# Autodesk Inventor assembly: Assembly1
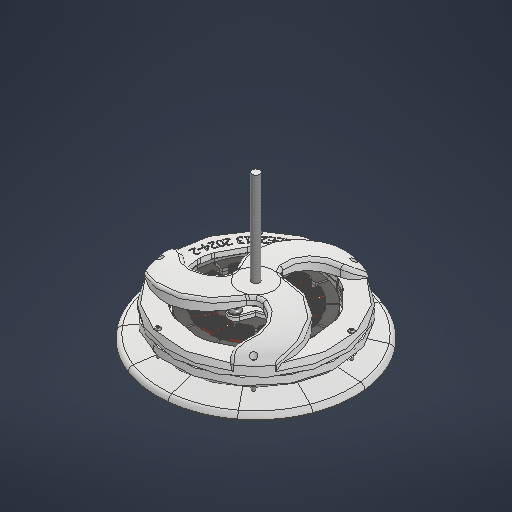
[picture p0: Inventor's stored thumbnail of the model, 512x512]
Saved by Autodesk Inventor 2025 (Build 290162010, 162A)
## iProperties
Created: 2024-11-09
Part Number: Assembly1
Document SubType Name: Assembly
Designer: river
Author: river
## Documents named in this file (15)
- C:\DATA\sem_08\Maquinas\proyecto\3d\Assembly1.iam
- C:\DATA\sem_08\Maquinas\proyecto\3d\lamina_estator.ipt
- C:\Users\river\Documents\Inventor\Content Center Files\R2025\en-US\DIN 625 SKF(4)\DIN 625 SKF - SKF 608-2Z.ipt
- C:\DATA\sem_08\Maquinas\proyecto\3d\perno.ipt
- C:\DATA\sem_08\Maquinas\proyecto\3d\lamina_rotor.ipt
- C:\DATA\sem_08\Maquinas\proyecto\3d\iman.ipt
- C:\DATA\sem_08\Maquinas\proyecto\3d\coil.ipt
- C:\DATA\sem_08\Maquinas\proyecto\3d\shell_b.ipt
- C:\DATA\sem_08\Maquinas\proyecto\3d\shell_t.ipt
- C:\Users\river\Documents\Inventor\Content Center Files\R2025\en-US\ANSI B18.3.4M(2)\ANSI B18.3.4M - M6 x 1 x 30(1).ipt
- C:\Users\river\Documents\Inventor\Content Center Files\R2025\en-US\ANSI B18.16.3M(2)\ANSI B18.16.3M - Property Class 5 and 10 - Metric M6 x 1 Metal Type.ipt
- C:\DATA\sem_08\Maquinas\proyecto\3d\rodamiento_t.ipt
- C:\DATA\sem_08\Maquinas\proyecto\3d\rodamiento_b.ipt
- C:\Users\river\Documents\Inventor\Content Center Files\R2025\en-US\ANSI B18.3.4M(2)\ANSI B18.3.4M - M3 x 0.5 x 25(1).ipt
- C:\Users\river\Documents\Inventor\Content Center Files\R2025\en-US\JIS B 1181 F C (1)\JIS B 1181 - M3(7).ipt
## Components (55 placed, 14 different names)
1. rodamiento_b:1 — Insert:19, Cylindrical:1, Insert:21
2. lamina_estator:1 — Mate:1, Mate:2, Flush:1, Insert:1, Flush:2
3. lamina_estator:2 — Insert:1, Flush:2, Insert:2, Flush:3, Mate:7
4. lamina_estator:3 — Insert:2, Flush:3, Insert:4, Insert:5, Insert:10, Mate:9
5. DIN 625 SKF- with two Z shields SKF 608-2Z:1 — Insert:3, Insert:9
6. DIN 625 SKF- with two Z shields SKF 608-2Z:2 — Insert:3, Insert:8
7. rodamiento_t:1 — Insert:4, Insert:5, Insert:8, Insert:14, Insert:19
8. perno:1 — Insert:9
9. lamina_rotor:1 — Mate:3, Flush:4, Flush:5, Insert:16, Mate:10
10. lamina_rotor:2 — Mate:3, Flush:4, Flush:5, Mate:4, Flush:6, Flush:7, Mate:5, Mate:6
11. lamina_rotor:3 — Mate:4, Flush:6, Flush:7, Insert:10
12. shell_t:1 — Insert:17, Insert:18, Insert:22
13. shell_b:1 — Insert:16, Mate:10, Insert:17, Insert:18, Insert:23
14. Prevailing Torque Type Hex Nut - Steel Metric Property Class 5 and 10 - Metric M6 x 1 Metal Type:1 — Insert:21
15. Forged Hexagon Socket Button Head Cap Screw - Metric M6 x 1 x 30:1 — Insert:14, Cylindrical:1
16. Prevailing Torque Type Hex Nut - Steel Metric Property Class 5 and 10 - Metric M6 x 1 Metal Type:2
17. Forged Hexagon Socket Button Head Cap Screw - Metric M6 x 1 x 30:2
18. Prevailing Torque Type Hex Nut - Steel Metric Property Class 5 and 10 - Metric M6 x 1 Metal Type:3
19. Forged Hexagon Socket Button Head Cap Screw - Metric M6 x 1 x 30:3
20. Prevailing Torque Type Hex Nut - Steel Metric Property Class 5 and 10 - Metric M6 x 1 Metal Type:4
21. Forged Hexagon Socket Button Head Cap Screw - Metric M6 x 1 x 30:4
22. Forged Hexagon Socket Button Head Cap Screw - Metric M3 x 0.5 x 25:1 — Insert:22
23. Forged Hexagon Socket Button Head Cap Screw - Metric M3 x 0.5 x 25:2
24. Forged Hexagon Socket Button Head Cap Screw - Metric M3 x 0.5 x 25:3
25. Forged Hexagon Socket Button Head Cap Screw - Metric M3 x 0.5 x 25:4
26. Forged Hexagon Socket Button Head Cap Screw - Metric M3 x 0.5 x 25:5
27. Forged Hexagon Socket Button Head Cap Screw - Metric M3 x 0.5 x 25:6
28. JIS B 1181 -finished Class 1 - Metric Class 1 -finishedM3:1 — Insert:23
29. JIS B 1181 -finished Class 1 - Metric Class 1 -finishedM3:2
30. JIS B 1181 -finished Class 1 - Metric Class 1 -finishedM3:3
31. JIS B 1181 -finished Class 1 - Metric Class 1 -finishedM3:4
32. JIS B 1181 -finished Class 1 - Metric Class 1 -finishedM3:5
33. JIS B 1181 -finished Class 1 - Metric Class 1 -finishedM3:6
34. coil:1 — Mate:7, Mate:9
35. coil:2
36. coil:3
37. coil:4
38. coil:5
39. coil:6
40. coil:7
41. coil:8
42. coil:9
43. coil:10
44. coil:11
45. coil:12
46. iman:1 — Mate:5, Mate:6
47. iman:2
48. iman:3
49. iman:4
50. iman:5
51. iman:6
52. iman:7
53. iman:8
54. iman:9
55. iman:10
## Component patterns: (4 elements, first: Prevailing Torque Type Hex Nut - Steel Metric Property Class 5 and 10 - Metric M6 x 1 Metal Type:1 + Forged Hexagon Socket Button Head Cap Screw - Metric M6 x 1 x 30:1), (6 elements, first: Forged Hexagon Socket Button Head Cap Screw - Metric M3 x 0.5 x 25:1), (6 elements, first: JIS B 1181 -finished Class 1 - Metric Class 1 -finishedM3:1), (12 elements, first: coil:1), (10 elements, first: iman:1)
## Relationships (33: Insert 16, Mate 9, Flush 7, CylindricalJoint 1)
- Mate:1: lamina_estator:1
- Mate:2: lamina_estator:1
- Flush:1: lamina_estator:1
- Insert:1: lamina_estator:1 ↔ lamina_estator:2
- Flush:2: lamina_estator:1 ↔ lamina_estator:2
- Insert:2: lamina_estator:2 ↔ lamina_estator:3
- Flush:3: lamina_estator:2 ↔ lamina_estator:3
- Insert:3: DIN 625 SKF- with two Z shields SKF 608-2Z:1 ↔ DIN 625 SKF- with two Z shields SKF 608-2Z:2
- Insert:4: lamina_estator:3 ↔ rodamiento_t:1
- Insert:5: lamina_estator:3 ↔ rodamiento_t:1
- Insert:8: DIN 625 SKF- with two Z shields SKF 608-2Z:2 ↔ rodamiento_t:1
- Insert:9: DIN 625 SKF- with two Z shields SKF 608-2Z:1 ↔ perno:1
- Mate:3: lamina_rotor:1 ↔ lamina_rotor:2
- Flush:4: lamina_rotor:1 ↔ lamina_rotor:2
- Flush:5: lamina_rotor:1 ↔ lamina_rotor:2
- Mate:4: lamina_rotor:2 ↔ lamina_rotor:3
- Flush:6: lamina_rotor:2 ↔ lamina_rotor:3
- Flush:7: lamina_rotor:2 ↔ lamina_rotor:3
- Insert:10: lamina_estator:3 ↔ lamina_rotor:3
- Mate:5: lamina_rotor:2 ↔ iman:1
- Mate:6: lamina_rotor:2 ↔ iman:1
- Mate:7: lamina_estator:2 ↔ coil:1
- Mate:9: lamina_estator:3 ↔ coil:1
- Insert:14: rodamiento_t:1 ↔ Forged Hexagon Socket Button Head Cap Screw - Metric M6 x 1 x 30:1
- Insert:16: lamina_rotor:1 ↔ shell_b:1
- Mate:10: lamina_rotor:1 ↔ shell_b:1
- Insert:17: shell_t:1 ↔ shell_b:1
- Insert:18: shell_t:1 ↔ shell_b:1
- Insert:19: rodamiento_b:1 ↔ rodamiento_t:1
- Cylindrical:1: rodamiento_b:1 ↔ Forged Hexagon Socket Button Head Cap Screw - Metric M6 x 1 x 30:1
- Insert:21: rodamiento_b:1 ↔ Prevailing Torque Type Hex Nut - Steel Metric Property Class 5 and 10 - Metric M6 x 1 Metal Type:1
- Insert:22: shell_t:1 ↔ Forged Hexagon Socket Button Head Cap Screw - Metric M3 x 0.5 x 25:1
- Insert:23: shell_b:1 ↔ JIS B 1181 -finished Class 1 - Metric Class 1 -finishedM3:1
